# Autodesk Inventor assembly: camaravision
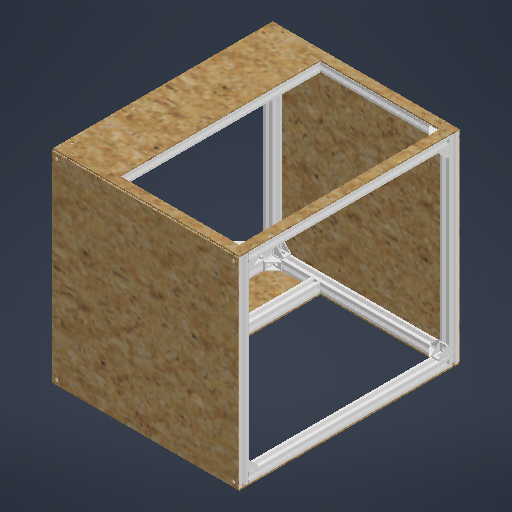
[picture p0: Inventor's stored thumbnail of the model, 512x512]
Saved by Autodesk Inventor 2026.2 (Build 302298010, 298A)
## iProperties
Created: 2026-04-14
Part Number: camaravision
Document SubType Name: Assembly
Designer: grego
Author: grego
## Documents named in this file (7)
- C:\Users\grego\OneDrive\Escritorio\PDM\camaravision.iam
- C:\Users\grego\OneDrive\Escritorio\PDM\VSLOT20x20x400.ipt
- C:\Users\grego\OneDrive\Escritorio\PDM\VSLOT20x20x420.ipt
- C:\Users\grego\OneDrive\Escritorio\PDM\VSLOT20x20x350.ipt
- C:\Users\grego\OneDrive\Escritorio\PDM\ANGULOESQUINA.ipt
- C:\Users\grego\OneDrive\Escritorio\PDM\TapaLateral.ipt
- C:\Users\grego\OneDrive\Escritorio\PDM\TapaFrontal.ipt
## Components (36 placed, 6 different names)
1. VSLOT20x20x400:1 — Mate:1, Flush:1, Flush:2, Mate:5, Flush:9, Flush:10, Mate:6, Flush:11, Flush:12, Mate:16, Mate:18, Mate:26, Mate:27, Flush:26
2. VSLOT20x20x420:1 — Mate:1, Flush:1, Flush:2, Mate:2, Flush:3, Flush:4, Mate:25, Mate:29, Mate:39, Mate:41
3. VSLOT20x20x400:2 — Mate:2, Flush:3, Flush:4, Mate:3, Flush:5, Flush:6, Mate:4, Flush:7, Flush:8, Mate:7, Flush:13, Flush:14, Mate:34, Mate:35, Mate:38, Mate:40
4. VSLOT20x20x420:2 — Mate:3, Flush:5, Flush:6, Mate:14, Mate:15, Mate:31, Mate:36, Flush:28
5. VSLOT20x20x350:1 — Mate:4, Flush:7, Flush:8, Mate:37, Mate:42, Flush:29, Mate:56
6. VSLOT20x20x350:2 — Mate:7, Flush:13, Flush:14, Mate:8, Mate:9, Flush:15, Flush:16, Mate:32, Mate:33, Flush:23, Flush:27, Mate:54
7. VSLOT20x20x350:3 — Mate:6, Flush:11, Flush:12, Mate:10, Flush:17, Flush:18, Mate:13, Mate:17, Mate:20, Mate:23, Flush:25
8. VSLOT20x20x350:4 — Mate:5, Flush:9, Flush:10, Mate:28, Mate:30, Mate:46, Mate:47
9. VSLOT20x20x420:3 — Mate:10, Flush:17, Flush:18, Mate:11, Flush:19, Flush:20, Mate:12, Flush:21, Flush:22, Mate:21, Mate:24, Mate:44, Mate:45, Mate:50
10. VSLOT20x20x420:4 — Mate:8, Mate:9, Flush:15, Flush:16, Mate:49, Flush:24
11. VSLOT20x20x400:3 — Mate:11, Flush:19, Flush:20, Mate:19, Mate:22, Mate:51
12. VSLOT20x20x400:4 — Mate:12, Flush:21, Flush:22, Mate:43, Mate:48, Mate:52, Flush:30
13. ANGULOESQUINA:1 — Mate:13, Mate:14
14. ANGULOESQUINA:2 — Mate:17, Mate:18
15. ANGULOESQUINA:4 — Mate:31, Mate:32
16. ANGULOESQUINA:5 — Mate:25, Mate:26
17. ANGULOESQUINA:7 — Mate:35, Mate:36
18. ANGULOESQUINA:8 — Mate:47, Mate:48
19. ANGULOESQUINA:9 — Mate:37, Mate:38
20. ANGULOESQUINA:11 — Mate:45, Mate:46
21. ANGULOESQUINA:12 — Mate:43, Mate:44
22. ANGULOESQUINA:13 — Mate:19, Mate:20
23. ANGULOESQUINA:14 — Mate:23, Mate:24
24. ANGULOESQUINA:15 — Mate:21, Mate:22
25. ANGULOESQUINA:16 — Mate:15, Mate:16
26. ANGULOESQUINA:17 — Mate:27, Mate:28
27. ANGULOESQUINA:18 — Mate:29, Mate:30
28. ANGULOESQUINA:19 — Mate:41, Mate:42
29. ANGULOESQUINA:21 — Mate:33, Mate:34
30. ANGULOESQUINA:22 — Mate:39, Mate:40
31. TapaLateral:1 — Mate:49, Flush:23, Flush:24
32. TapaLateral:2 — Mate:50, Flush:25, Flush:26
33. VSLOT20x20x400:5 — Mate:53, Mate:54, Flush:31
34. TapaFrontal:1 — Mate:51, Flush:27, Flush:28, Mate:53, Flush:31
35. TapaFrontal:2 — Mate:52, Flush:29, Flush:30, Mate:55, Flush:32
36. VSLOT20x20x420:5 — Mate:55, Mate:56, Flush:32
## Relationships (88: Mate 56, Flush 32)
- Mate:1: VSLOT20x20x400:1 ↔ VSLOT20x20x420:1
- Flush:1: VSLOT20x20x400:1 ↔ VSLOT20x20x420:1
- Flush:2: VSLOT20x20x400:1 ↔ VSLOT20x20x420:1
- Mate:2: VSLOT20x20x420:1 ↔ VSLOT20x20x400:2
- Flush:3: VSLOT20x20x420:1 ↔ VSLOT20x20x400:2
- Flush:4: VSLOT20x20x420:1 ↔ VSLOT20x20x400:2
- Mate:3: VSLOT20x20x400:2 ↔ VSLOT20x20x420:2
- Flush:5: VSLOT20x20x400:2 ↔ VSLOT20x20x420:2
- Flush:6: VSLOT20x20x400:2 ↔ VSLOT20x20x420:2
- Mate:4: VSLOT20x20x400:2 ↔ VSLOT20x20x350:1
- Flush:7: VSLOT20x20x400:2 ↔ VSLOT20x20x350:1
- Flush:8: VSLOT20x20x400:2 ↔ VSLOT20x20x350:1
- Mate:5: VSLOT20x20x400:1 ↔ VSLOT20x20x350:4
- Flush:9: VSLOT20x20x400:1 ↔ VSLOT20x20x350:4
- Flush:10: VSLOT20x20x400:1 ↔ VSLOT20x20x350:4
- Mate:6: VSLOT20x20x400:1 ↔ VSLOT20x20x350:3
- Flush:11: VSLOT20x20x400:1 ↔ VSLOT20x20x350:3
- Flush:12: VSLOT20x20x400:1 ↔ VSLOT20x20x350:3
- Mate:7: VSLOT20x20x400:2 ↔ VSLOT20x20x350:2
- Flush:13: VSLOT20x20x400:2 ↔ VSLOT20x20x350:2
- Flush:14: VSLOT20x20x400:2 ↔ VSLOT20x20x350:2
- Mate:8: VSLOT20x20x350:2 ↔ VSLOT20x20x420:4
- Mate:9: VSLOT20x20x350:2 ↔ VSLOT20x20x420:4
- Flush:15: VSLOT20x20x350:2 ↔ VSLOT20x20x420:4
- Flush:16: VSLOT20x20x350:2 ↔ VSLOT20x20x420:4
- Mate:10: VSLOT20x20x350:3 ↔ VSLOT20x20x420:3
- Flush:17: VSLOT20x20x350:3 ↔ VSLOT20x20x420:3
- Flush:18: VSLOT20x20x350:3 ↔ VSLOT20x20x420:3
- Mate:11: VSLOT20x20x420:3 ↔ VSLOT20x20x400:3
- Flush:19: VSLOT20x20x420:3 ↔ VSLOT20x20x400:3
- Flush:20: VSLOT20x20x420:3 ↔ VSLOT20x20x400:3
- Mate:12: VSLOT20x20x420:3 ↔ VSLOT20x20x400:4
- Flush:21: VSLOT20x20x420:3 ↔ VSLOT20x20x400:4
- Flush:22: VSLOT20x20x420:3 ↔ VSLOT20x20x400:4
- Mate:13: VSLOT20x20x350:3 ↔ ANGULOESQUINA:1
- Mate:14: VSLOT20x20x420:2 ↔ ANGULOESQUINA:1
- Mate:15: VSLOT20x20x420:2 ↔ ANGULOESQUINA:16
- Mate:16: VSLOT20x20x400:1 ↔ ANGULOESQUINA:16
- Mate:17: VSLOT20x20x350:3 ↔ ANGULOESQUINA:2
- Mate:18: VSLOT20x20x400:1 ↔ ANGULOESQUINA:2
- Mate:19: VSLOT20x20x400:3 ↔ ANGULOESQUINA:13
- Mate:20: VSLOT20x20x350:3 ↔ ANGULOESQUINA:13
- Mate:21: VSLOT20x20x420:3 ↔ ANGULOESQUINA:15
- Mate:22: VSLOT20x20x400:3 ↔ ANGULOESQUINA:15
- Mate:23: VSLOT20x20x350:3 ↔ ANGULOESQUINA:14
- Mate:24: VSLOT20x20x420:3 ↔ ANGULOESQUINA:14
- Mate:25: VSLOT20x20x420:1 ↔ ANGULOESQUINA:5
- Mate:26: VSLOT20x20x400:1 ↔ ANGULOESQUINA:5
- Mate:27: VSLOT20x20x400:1 ↔ ANGULOESQUINA:17
- Mate:28: VSLOT20x20x350:4 ↔ ANGULOESQUINA:17
- Mate:29: VSLOT20x20x420:1 ↔ ANGULOESQUINA:18
- Mate:30: VSLOT20x20x350:4 ↔ ANGULOESQUINA:18
- Mate:31: VSLOT20x20x420:2 ↔ ANGULOESQUINA:4
- Mate:32: VSLOT20x20x350:2 ↔ ANGULOESQUINA:4
- Mate:33: VSLOT20x20x350:2 ↔ ANGULOESQUINA:21
- Mate:34: VSLOT20x20x400:2 ↔ ANGULOESQUINA:21
- Mate:35: VSLOT20x20x400:2 ↔ ANGULOESQUINA:7
- Mate:36: VSLOT20x20x420:2 ↔ ANGULOESQUINA:7
- Mate:37: VSLOT20x20x350:1 ↔ ANGULOESQUINA:9
- Mate:38: VSLOT20x20x400:2 ↔ ANGULOESQUINA:9
- Mate:39: VSLOT20x20x420:1 ↔ ANGULOESQUINA:22
- Mate:40: VSLOT20x20x400:2 ↔ ANGULOESQUINA:22
- Mate:41: VSLOT20x20x420:1 ↔ ANGULOESQUINA:19
- Mate:42: VSLOT20x20x350:1 ↔ ANGULOESQUINA:19
- Mate:43: VSLOT20x20x400:4 ↔ ANGULOESQUINA:12
- Mate:44: VSLOT20x20x420:3 ↔ ANGULOESQUINA:12
- Mate:45: VSLOT20x20x420:3 ↔ ANGULOESQUINA:11
- Mate:46: VSLOT20x20x350:4 ↔ ANGULOESQUINA:11
- Mate:47: VSLOT20x20x350:4 ↔ ANGULOESQUINA:8
- Mate:48: VSLOT20x20x400:4 ↔ ANGULOESQUINA:8
- Mate:49: VSLOT20x20x420:4 ↔ TapaLateral:1
- Flush:23: VSLOT20x20x350:2 ↔ TapaLateral:1
- Flush:24: VSLOT20x20x420:4 ↔ TapaLateral:1
- Mate:50: VSLOT20x20x420:3 ↔ TapaLateral:2
- Flush:25: VSLOT20x20x350:3 ↔ TapaLateral:2
- Flush:26: VSLOT20x20x400:1 ↔ TapaLateral:2
- Mate:51: VSLOT20x20x400:3 ↔ TapaFrontal:1
- Flush:27: VSLOT20x20x350:2 ↔ TapaFrontal:1
- Flush:28: VSLOT20x20x420:2 ↔ TapaFrontal:1
- Mate:52: VSLOT20x20x400:4 ↔ TapaFrontal:2
- Flush:29: VSLOT20x20x350:1 ↔ TapaFrontal:2
- Flush:30: VSLOT20x20x400:4 ↔ TapaFrontal:2
- Mate:53: VSLOT20x20x400:5 ↔ TapaFrontal:1
- Mate:54: VSLOT20x20x350:2 ↔ VSLOT20x20x400:5
- Flush:31: VSLOT20x20x400:5 ↔ TapaFrontal:1
- Mate:55: TapaFrontal:2 ↔ VSLOT20x20x420:5
- Mate:56: VSLOT20x20x350:1 ↔ VSLOT20x20x420:5
- Flush:32: TapaFrontal:2 ↔ VSLOT20x20x420:5
